# Autodesk Inventor assembly: Reducer
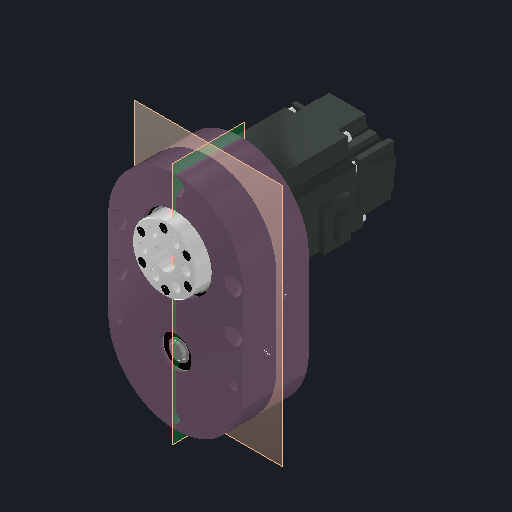
[picture p0: Inventor's stored thumbnail of the model, 512x512]
Saved by Autodesk Inventor 2026 (Build 300175000, 175)
## iProperties
Created: 2025-11-29
Part Number: Reducer
Document SubType Name: Assembly
Designer: pochi
Mass: 1517.22 g
Surface Area: 1876.83 cm^2
Volume: 564.379 cm^3
Density: 2.6883 g/cm^3
Author: pochi
## Documents named in this file (25)
- D:\POLIMI\3RD SEMESTER\Industrial Robotics\Project\Mine\Reducer.iam
- D:\POLIMI\3RD SEMESTER\Industrial Robotics\Project\Mine\Housing.ipt
- D:\POLIMI\3RD SEMESTER\Industrial Robotics\Project\Mine\Bearing_01.ipt
- D:\POLIMI\3RD SEMESTER\Industrial Robotics\Project\Mine\Shaft_01.ipt
- D:\POLIMI\3RD SEMESTER\Industrial Robotics\Project\Mine\Spacer_01.ipt
- D:\POLIMI\3RD SEMESTER\Industrial Robotics\Project\Mine\Motor_02.ipt
- D:\POLIMI\3RD SEMESTER\Industrial Robotics\Project\Mine\Spacer_03.ipt
- D:\POLIMI\3RD SEMESTER\Industrial Robotics\Project\Mine\Pulley_3M20T.ipt
- D:\POLIMI\3RD SEMESTER\Industrial Robotics\Project\Mine\Pulley_3M40T.ipt
- D:\POLIMI\3RD SEMESTER\Industrial Robotics\Project\Mine\Belt_01.ipt
- D:\POLIMI\3RD SEMESTER\Industrial Robotics\Project\Mine\Spacer_02.ipt
- D:\POLIMI\3RD SEMESTER\Industrial Robotics\Project\Mine\Pulley_3M20T_02.ipt
- D:\POLIMI\3RD SEMESTER\Industrial Robotics\Project\Mine\Bearing_02.ipt
- D:\POLIMI\3RD SEMESTER\Industrial Robotics\Project\Mine\Pulley_3M40T_02.ipt
- D:\POLIMI\3RD SEMESTER\Industrial Robotics\Project\Mine\Belt_02.ipt
- D:\POLIMI\3RD SEMESTER\Industrial Robotics\Project\Mine\Spacer_04.ipt
- D:\POLIMI\3RD SEMESTER\Industrial Robotics\Project\Mine\ActuationDisk.ipt
- D:\POLIMI\3RD SEMESTER\Industrial Robotics\Project\Mine\M3_Screw.ipt
- D:\POLIMI\3RD SEMESTER\Industrial Robotics\Project\Mine\Bearing_03.ipt
- D:\POLIMI\3RD SEMESTER\Industrial Robotics\Project\Mine\Cover.ipt
- D:\POLIMI\3RD SEMESTER\Industrial Robotics\Project\Mine\Bearing_Tension_01.ipt
- D:\POLIMI\3RD SEMESTER\Industrial Robotics\Project\Mine\Tensioning_01.ipt
- D:\POLIMI\3RD SEMESTER\Industrial Robotics\Project\Mine\New_Belt_01.ipt
- D:\POLIMI\3RD SEMESTER\Industrial Robotics\Project\Mine\New_Belt_02.ipt
- D:\POLIMI\3RD SEMESTER\Industrial Robotics\Project\Mine\Spring_Tesion.ipt
## Components (36 placed, 24 different names)
1. Housing:1 — Mate:122, Mate:123, Flush:16, Mate:127, Mate:128, Mate:129, Symmetry:1, Symmetry:2, Mate:178, Mate:183, Cylindrical:1
2. Bearing_01:1 — Mate:122, Mate:123, Mate:124, Mate:126
3. Shaft_01:1 — Flush:16, Mate:124, Mate:125, Mate:134, Mate:141, Mate:143, Mate:152, Mate:154
4. Spacer_01:1 — Mate:125, Mate:126, Mate:135
5. Motor_02:1 — Mate:127, Mate:128, Mate:129, Mate:130, Mate:131, Mate:132, Mate:139, Mate:145
6. Spacer_03:1 — Mate:130, Mate:131, Mate:133
7. Pulley_3M20T:1 — Mate:132, Mate:133, Mate:137, Mate:140, Mate:180, Mate:181
8. Pulley_3M40T:1 — Mate:134, Mate:135, Mate:136, Mate:138, Mate:142, Mate:179
9. Belt_01:1 — Mate:136, Mate:137, Mate:138
10. Spacer_02:1 — Mate:139, Mate:140, Mate:146
11. Spacer_01:2 — Mate:141, Mate:142, Mate:144
12. Pulley_3M20T_02:1 — Mate:143, Mate:144, Mate:151, Mate:153, Mate:185, Mate:186
13. Bearing_02:1 — Mate:145, Mate:146, Mate:147, Mate:148
14. Pulley_3M40T_02:1 — Mate:147, Mate:148, Mate:149, Mate:150, Mate:156, Mate:157, Mate:158, Mate:184
15. Belt_02:1 — Mate:149, Mate:150, Mate:151
16. Spacer_04:1 — Mate:152, Mate:153, Mate:155
17. Bearing_01:2 — Mate:154, Mate:155, Mate:167, Mate:168
18. ActuationDisk:1 — Mate:156, Mate:157, Mate:158, Flush:17, Mate:159, Flush:18, Mate:160, Flush:19, Mate:161, Flush:20, Mate:162, Flush:21, Mate:163, Flush:22, Mate:164, Mate:165, Mate:166, Cylindrical:1
19. M3_Screw:1 — Flush:17, Mate:159
20. M3_Screw:2 — Flush:18, Mate:160
21. M3_Screw:3 — Flush:19, Mate:161
22. M3_Screw:4 — Flush:20, Mate:162
23. M3_Screw:5 — Flush:21, Mate:163
24. M3_Screw:6 — Flush:22, Mate:164
25. Bearing_03:1 — Mate:165, Mate:166, Mate:169
26. Cover:1 — Mate:167, Mate:168, Mate:169, Symmetry:1, Symmetry:2
27. Bearing_Tension_01:1 — Mate:172, Mate:173
28. Tensioning_01:1 — Mate:174, Mate:175, Mate:183, Mate:188, Mate:189
29. Tensioning_01:2 — Mate:170, Mate:171, Mate:173, Mate:178, Mate:190, Mate:191
30. Bearing_Tension_01:2 — Mate:176, Mate:177, Mate:187
31. Bearing_Tension_01:3 — Mate:170, Mate:171, Mate:172, Mate:182
32. Bearing_Tension_01:4 — Mate:174, Mate:175, Mate:176, Mate:177
33. New_Belt_01:1 — Mate:179, Mate:180, Mate:181, Mate:182
34. New_Belt_02:1 — Mate:184, Mate:185, Mate:186, Mate:187
35. Spring_Tesion:1 — Mate:188, Mate:189
36. Spring_Tesion:2 — Mate:190, Mate:191
## Relationships (80: Mate 70, Flush 7, Symmetry 2, CylindricalJoint 1)
- Mate:122: Housing:1 ↔ Bearing_01:1
- Mate:123: Housing:1 ↔ Bearing_01:1
- Flush:16: Housing:1 ↔ Shaft_01:1
- Mate:124: Bearing_01:1 ↔ Shaft_01:1
- Mate:125: Shaft_01:1 ↔ Spacer_01:1
- Mate:126: Bearing_01:1 ↔ Spacer_01:1
- Mate:127: Housing:1 ↔ Motor_02:1
- Mate:128: Housing:1 ↔ Motor_02:1
- Mate:129: Housing:1 ↔ Motor_02:1
- Mate:130: Motor_02:1 ↔ Spacer_03:1
- Mate:131: Motor_02:1 ↔ Spacer_03:1
- Mate:132: Motor_02:1 ↔ Pulley_3M20T:1
- Mate:133: Spacer_03:1 ↔ Pulley_3M20T:1
- Mate:134: Shaft_01:1 ↔ Pulley_3M40T:1
- Mate:135: Spacer_01:1 ↔ Pulley_3M40T:1
- Mate:136: Pulley_3M40T:1 ↔ Belt_01:1
- Mate:137: Pulley_3M20T:1 ↔ Belt_01:1
- Mate:138: Pulley_3M40T:1 ↔ Belt_01:1
- Mate:139: Motor_02:1 ↔ Spacer_02:1
- Mate:140: Pulley_3M20T:1 ↔ Spacer_02:1
- Mate:141: Shaft_01:1 ↔ Spacer_01:2
- Mate:142: Pulley_3M40T:1 ↔ Spacer_01:2
- Mate:143: Shaft_01:1 ↔ Pulley_3M20T_02:1
- Mate:144: Spacer_01:2 ↔ Pulley_3M20T_02:1
- Mate:145: Motor_02:1 ↔ Bearing_02:1
- Mate:146: Spacer_02:1 ↔ Bearing_02:1
- Mate:147: Bearing_02:1 ↔ Pulley_3M40T_02:1
- Mate:148: Bearing_02:1 ↔ Pulley_3M40T_02:1
- Mate:149: Pulley_3M40T_02:1 ↔ Belt_02:1
- Mate:150: Pulley_3M40T_02:1 ↔ Belt_02:1
- Mate:151: Pulley_3M20T_02:1 ↔ Belt_02:1
- Mate:152: Shaft_01:1 ↔ Spacer_04:1
- Mate:153: Pulley_3M20T_02:1 ↔ Spacer_04:1
- Mate:154: Shaft_01:1 ↔ Bearing_01:2
- Mate:155: Spacer_04:1 ↔ Bearing_01:2
- Mate:156: Pulley_3M40T_02:1 ↔ ActuationDisk:1
- Mate:157: Pulley_3M40T_02:1 ↔ ActuationDisk:1
- Mate:158: Pulley_3M40T_02:1 ↔ ActuationDisk:1
- Flush:17: ActuationDisk:1 ↔ M3_Screw:1
- Mate:159: ActuationDisk:1 ↔ M3_Screw:1
- Flush:18: ActuationDisk:1 ↔ M3_Screw:2
- Mate:160: ActuationDisk:1 ↔ M3_Screw:2
- Flush:19: ActuationDisk:1 ↔ M3_Screw:3
- Mate:161: ActuationDisk:1 ↔ M3_Screw:3
- Flush:20: ActuationDisk:1 ↔ M3_Screw:4
- Mate:162: ActuationDisk:1 ↔ M3_Screw:4
- Flush:21: ActuationDisk:1 ↔ M3_Screw:5
- Mate:163: ActuationDisk:1 ↔ M3_Screw:5
- Flush:22: ActuationDisk:1 ↔ M3_Screw:6
- Mate:164: ActuationDisk:1 ↔ M3_Screw:6
- Mate:165: ActuationDisk:1 ↔ Bearing_03:1
- Mate:166: ActuationDisk:1 ↔ Bearing_03:1
- Mate:167: Bearing_01:2 ↔ Cover:1
- Mate:168: Bearing_01:2 ↔ Cover:1
- Mate:169: Bearing_03:1 ↔ Cover:1
- Symmetry:1: Housing:1 ↔ Cover:1
- Symmetry:2: Housing:1 ↔ Cover:1
- Mate:170: Tensioning_01:2 ↔ Bearing_Tension_01:3
- Mate:171: Tensioning_01:2 ↔ Bearing_Tension_01:3
- Mate:172: Bearing_Tension_01:1 ↔ Bearing_Tension_01:3
- Mate:173: Bearing_Tension_01:1 ↔ Tensioning_01:2
- Mate:174: Tensioning_01:1 ↔ Bearing_Tension_01:4
- Mate:175: Tensioning_01:1 ↔ Bearing_Tension_01:4
- Mate:176: Bearing_Tension_01:2 ↔ Bearing_Tension_01:4
- Mate:177: Bearing_Tension_01:2 ↔ Bearing_Tension_01:4
- Mate:178: Housing:1 ↔ Tensioning_01:2
- Mate:179: Pulley_3M40T:1 ↔ New_Belt_01:1
- Mate:180: Pulley_3M20T:1 ↔ New_Belt_01:1
- Mate:181: Pulley_3M20T:1 ↔ New_Belt_01:1
- Mate:182: Bearing_Tension_01:3 ↔ New_Belt_01:1
- Mate:183: Housing:1 ↔ Tensioning_01:1
- Mate:184: Pulley_3M40T_02:1 ↔ New_Belt_02:1
- Mate:185: Pulley_3M20T_02:1 ↔ New_Belt_02:1
- Mate:186: Pulley_3M20T_02:1 ↔ New_Belt_02:1
- Mate:187: Bearing_Tension_01:2 ↔ New_Belt_02:1
- Mate:188: Tensioning_01:1 ↔ Spring_Tesion:1
- Mate:189: Tensioning_01:1 ↔ Spring_Tesion:1
- Mate:190: Tensioning_01:2 ↔ Spring_Tesion:2
- Mate:191: Tensioning_01:2 ↔ Spring_Tesion:2
- Cylindrical:1: Housing:1 ↔ ActuationDisk:1
